# Autodesk Inventor assembly: MPPC
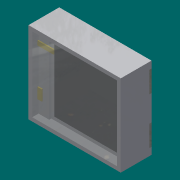
[picture p0: Inventor's stored thumbnail of the model, 180x180]
Saved by Autodesk Inventor 2016 SP1 (Build 200210100, 210)
## iProperties
Created: 2016-02-09
Part Number: MPPC
Document SubType Name: Assembly
Designer: Sawaiz
Author: Sawaiz
## Documents named in this file (3)
- C:\Users\sawai\OneDrive\projects\mppcSensorInterface\cad\electronics\mppc\MPPC.iam
- C:\Users\sawai\OneDrive\projects\mppcSensorInterface\cad\electronics\mppc\S13360.ipt
- C:\Users\sawai\OneDrive\projects\mppcSensorInterface\cad\electronics\mppc\lens.ipt
## Components (2 placed, 2 different names)
1. S13360:1 — Flush:1
2. lens:1 — Flush:1
## Relationships (1: Flush 1)
- Flush:1: S13360:1 ↔ lens:1
